# Autodesk Inventor assembly: CycloidalGearBoxAssemblyV1
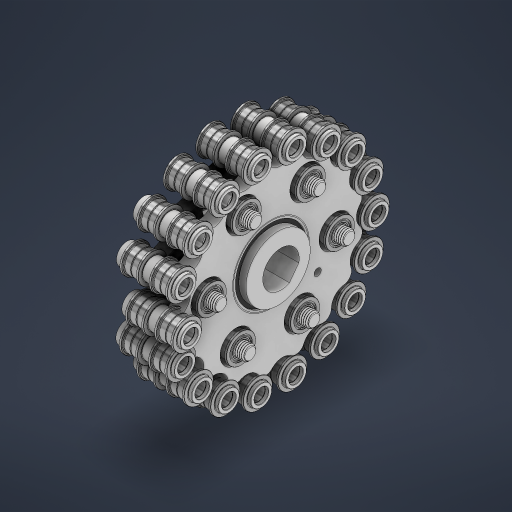
[picture p0: Inventor's stored thumbnail of the model, 512x512]
Saved by Autodesk Inventor 2024 (Build 280153000, 153)
## iProperties
Created: 2024-01-31
Part Number: CycloidalGearBoxAssemblyV1
Document SubType Name: Assembly
Designer: avsar
Author: avsar
## Documents named in this file (12)
- C:\Users\avsar\Documents\Inventor\RCR_Arm\Arm_V4\CycloidalGearBoxes\StageOneGearBox\CycloidalGearBoxAssemblyV1.iam
- C:\Users\avsar\Documents\Inventor\RCR_Arm\Arm_V4\CycloidalGearBoxes\StageOneGearBox\HousingFaceInput.ipt
- C:\Users\avsar\Documents\Inventor\RCR_Arm\Arm_V4\CycloidalGearBoxes\StageOneGearBox\Gearbox_MainBody.ipt
- C:\Users\avsar\Documents\Inventor\RCR_Arm\COTS\Motion\Bearings\Flanged Bearings\4x7x2.5mm Flanged Ball Bearing.ipt
- C:\Users\avsar\Documents\Inventor\RCR_Arm\COTS\ISO Standard Hardware\Spacers and Shims\4mm ID x 6mm OD Spacers\(1mm legnth) 4mm ID x 6mm OD Spacer.ipt
- C:\Users\avsar\Documents\Inventor\RCR_Arm\COTS\ISO Standard Hardware\Spacers and Shims\4mm ID x 6mm OD Spacers\(3mm legnth) 4mm ID x 6mm OD Spacer.ipt
- C:\Users\avsar\Documents\Inventor\RCR_Arm\Arm_V4\CycloidalGearBoxes\StageOneGearBox\RollerBearingShaft.ipt
- C:\Users\avsar\Documents\Inventor\RCR_Arm\Arm_V4\CycloidalGearBoxes\StageOneGearBox\CycloidalDisk.ipt
- C:\Users\avsar\Documents\Inventor\RCR_Arm\Arm_V4\CycloidalGearBoxes\StageOneGearBox\EccentricBearingShaft.ipt
- C:\Users\avsar\Documents\Inventor\RCR_Arm\COTS\Motion\Bearings\Standard Bearings\16mm ID x 22mm OD x 4mm Thickness Ball Bearing.ipt
- C:\Users\avsar\Documents\Inventor\RCR_Arm\COTS\ISO Standard Hardware\Screws\Sockethead Screws\Buttonhead Screws\M4 x 0.7mm\(M4 x 0.7 x 16) Sockethead Buttonhead Screw.ipt
- C:\Users\avsar\Documents\Inventor\RCR_Arm\Arm_V4\CycloidalGearBoxes\StageOneGearBox\HousingInputFaceSpacer.ipt
## Components (182 placed, 11 different names)
1. HousingFaceInput:1 — Mate:1, Mate:2, Mate:3, Mate:7, Mate:76, Mate:94, Mate:112, Mate:130, Mate:148, Mate:166, Mate:184, Mate:202, Mate:220, Mate:238, Mate:256, Mate:274, Mate:292, Mate:310, Mate:328, Mate:346, Mate:364
2. Gearbox_MainBody:1 — Mate:1, Mate:2, Mate:3
3. 4x7x2.5mm Flanged Ball Bearing:5 — Mate:10, Mate:11, Mate:12, Mate:13
4. RollerBearingShaft:2 — Mate:8, Mate:9, Mate:10, Mate:11
5. 4x7x2.5mm Flanged Ball Bearing:4 — Mate:7, Mate:8, Mate:9
6. (1mm legnth) 4mm ID x 6mm OD Spacer:2 — Mate:20, Mate:21
7. RollerBearingShaft:1 — Mate:16, Mate:17, Mate:18, Mate:19
8. 4x7x2.5mm Flanged Ball Bearing:2 — Mate:14, Mate:15, Mate:16, Mate:17
9. (3mm legnth) 4mm ID x 6mm OD Spacer:1 — Mate:12, Mate:13, Mate:14, Mate:15
10. 4x7x2.5mm Flanged Ball Bearing:1 — Mate:18, Mate:19, Mate:20, Mate:21
11. (1mm legnth) 4mm ID x 6mm OD Spacer:3 — Mate:76
12. 4x7x2.5mm Flanged Ball Bearing:6 — Mate:377
13. RollerBearingShaft:3
14. 4x7x2.5mm Flanged Ball Bearing:7
15. 4x7x2.5mm Flanged Ball Bearing:8
16. RollerBearingShaft:4
17. 4x7x2.5mm Flanged Ball Bearing:9
18. (3mm legnth) 4mm ID x 6mm OD Spacer:2
19. (1mm legnth) 4mm ID x 6mm OD Spacer:5 — Mate:94
20. 4x7x2.5mm Flanged Ball Bearing:10
21. RollerBearingShaft:5
22. 4x7x2.5mm Flanged Ball Bearing:11
23. 4x7x2.5mm Flanged Ball Bearing:12
24. RollerBearingShaft:6
25. 4x7x2.5mm Flanged Ball Bearing:13
26. (3mm legnth) 4mm ID x 6mm OD Spacer:3
27. (1mm legnth) 4mm ID x 6mm OD Spacer:7 — Mate:112
28. 4x7x2.5mm Flanged Ball Bearing:14
29. RollerBearingShaft:7
30. 4x7x2.5mm Flanged Ball Bearing:15 — Tangent:1
31. 4x7x2.5mm Flanged Ball Bearing:16
32. RollerBearingShaft:8
33. 4x7x2.5mm Flanged Ball Bearing:17
34. (3mm legnth) 4mm ID x 6mm OD Spacer:4
35. (1mm legnth) 4mm ID x 6mm OD Spacer:9
36. 4x7x2.5mm Flanged Ball Bearing:18
37. RollerBearingShaft:9
38. 4x7x2.5mm Flanged Ball Bearing:19
39. 4x7x2.5mm Flanged Ball Bearing:20 — Mate:130
40. RollerBearingShaft:10
41. 4x7x2.5mm Flanged Ball Bearing:21
42. (3mm legnth) 4mm ID x 6mm OD Spacer:5
43. (1mm legnth) 4mm ID x 6mm OD Spacer:11
44. 4x7x2.5mm Flanged Ball Bearing:22 — Mate:411, Mate:412
45. RollerBearingShaft:11
46. 4x7x2.5mm Flanged Ball Bearing:23
47. 4x7x2.5mm Flanged Ball Bearing:24 — Mate:148
48. RollerBearingShaft:12
49. 4x7x2.5mm Flanged Ball Bearing:25
50. (3mm legnth) 4mm ID x 6mm OD Spacer:6
51. (1mm legnth) 4mm ID x 6mm OD Spacer:13
52. 4x7x2.5mm Flanged Ball Bearing:26 — Mate:413, Mate:414
53. RollerBearingShaft:13
54. 4x7x2.5mm Flanged Ball Bearing:27 — Tangent:2
55. 4x7x2.5mm Flanged Ball Bearing:28 — Mate:166
56. RollerBearingShaft:14
57. 4x7x2.5mm Flanged Ball Bearing:29
58. (3mm legnth) 4mm ID x 6mm OD Spacer:7
59. (1mm legnth) 4mm ID x 6mm OD Spacer:15
60. 4x7x2.5mm Flanged Ball Bearing:30 — Mate:415, Mate:416
61. RollerBearingShaft:15
62. 4x7x2.5mm Flanged Ball Bearing:31
63. 4x7x2.5mm Flanged Ball Bearing:32 — Mate:184
64. RollerBearingShaft:16
65. 4x7x2.5mm Flanged Ball Bearing:33
66. (3mm legnth) 4mm ID x 6mm OD Spacer:8
67. (1mm legnth) 4mm ID x 6mm OD Spacer:17
68. 4x7x2.5mm Flanged Ball Bearing:34 — Mate:417, Mate:418
69. RollerBearingShaft:17
70. 4x7x2.5mm Flanged Ball Bearing:35
71. 4x7x2.5mm Flanged Ball Bearing:36 — Mate:202
72. RollerBearingShaft:18
73. 4x7x2.5mm Flanged Ball Bearing:37
74. (3mm legnth) 4mm ID x 6mm OD Spacer:9
75. (1mm legnth) 4mm ID x 6mm OD Spacer:19
76. 4x7x2.5mm Flanged Ball Bearing:38 — Mate:419, Mate:420
77. RollerBearingShaft:19
78. 4x7x2.5mm Flanged Ball Bearing:39
79. 4x7x2.5mm Flanged Ball Bearing:40 — Mate:220
80. RollerBearingShaft:20
81. 4x7x2.5mm Flanged Ball Bearing:41
82. (3mm legnth) 4mm ID x 6mm OD Spacer:10
83. (1mm legnth) 4mm ID x 6mm OD Spacer:21
84. 4x7x2.5mm Flanged Ball Bearing:42 — Mate:421, Mate:422
85. RollerBearingShaft:21
86. 4x7x2.5mm Flanged Ball Bearing:43
87. 4x7x2.5mm Flanged Ball Bearing:44 — Mate:238
88. RollerBearingShaft:22
89. 4x7x2.5mm Flanged Ball Bearing:45
90. (3mm legnth) 4mm ID x 6mm OD Spacer:11
91. (1mm legnth) 4mm ID x 6mm OD Spacer:23
92. 4x7x2.5mm Flanged Ball Bearing:46 — Mate:256, Mate:423, Mate:424
93. RollerBearingShaft:23
94. 4x7x2.5mm Flanged Ball Bearing:47
95. 4x7x2.5mm Flanged Ball Bearing:48
96. RollerBearingShaft:24
97. 4x7x2.5mm Flanged Ball Bearing:49
98. (3mm legnth) 4mm ID x 6mm OD Spacer:12
99. (1mm legnth) 4mm ID x 6mm OD Spacer:25
100. 4x7x2.5mm Flanged Ball Bearing:50 — Mate:425, Mate:426
101. RollerBearingShaft:25
102. 4x7x2.5mm Flanged Ball Bearing:51
103. 4x7x2.5mm Flanged Ball Bearing:52 — Mate:274
104. RollerBearingShaft:26
105. 4x7x2.5mm Flanged Ball Bearing:53
106. (3mm legnth) 4mm ID x 6mm OD Spacer:13
107. (1mm legnth) 4mm ID x 6mm OD Spacer:27
108. 4x7x2.5mm Flanged Ball Bearing:54 — Mate:427, Mate:428
109. RollerBearingShaft:27
110. 4x7x2.5mm Flanged Ball Bearing:55
111. 4x7x2.5mm Flanged Ball Bearing:56 — Mate:292
112. RollerBearingShaft:28
113. 4x7x2.5mm Flanged Ball Bearing:57
114. (3mm legnth) 4mm ID x 6mm OD Spacer:14
115. (1mm legnth) 4mm ID x 6mm OD Spacer:29
116. 4x7x2.5mm Flanged Ball Bearing:58 — Mate:429, Mate:430
117. RollerBearingShaft:29
118. 4x7x2.5mm Flanged Ball Bearing:59
119. 4x7x2.5mm Flanged Ball Bearing:60 — Mate:310
120. RollerBearingShaft:30
121. 4x7x2.5mm Flanged Ball Bearing:61
122. (3mm legnth) 4mm ID x 6mm OD Spacer:15
123. (1mm legnth) 4mm ID x 6mm OD Spacer:31
124. 4x7x2.5mm Flanged Ball Bearing:62 — Mate:431, Mate:432
125. RollerBearingShaft:31
126. 4x7x2.5mm Flanged Ball Bearing:63
127. 4x7x2.5mm Flanged Ball Bearing:64 — Mate:328
128. RollerBearingShaft:32
129. 4x7x2.5mm Flanged Ball Bearing:65
130. (3mm legnth) 4mm ID x 6mm OD Spacer:16
131. (1mm legnth) 4mm ID x 6mm OD Spacer:33
132. 4x7x2.5mm Flanged Ball Bearing:66 — Mate:433, Mate:434
133. RollerBearingShaft:33
134. 4x7x2.5mm Flanged Ball Bearing:67
135. 4x7x2.5mm Flanged Ball Bearing:68 — Mate:346
136. RollerBearingShaft:34
137. 4x7x2.5mm Flanged Ball Bearing:69
138. (3mm legnth) 4mm ID x 6mm OD Spacer:17
139. (1mm legnth) 4mm ID x 6mm OD Spacer:35
140. 4x7x2.5mm Flanged Ball Bearing:70 — Mate:435, Mate:436
141. RollerBearingShaft:35
142. 4x7x2.5mm Flanged Ball Bearing:71
143. 4x7x2.5mm Flanged Ball Bearing:72 — Mate:364, Tangent:15
144. RollerBearingShaft:36
145. 4x7x2.5mm Flanged Ball Bearing:73
146. (3mm legnth) 4mm ID x 6mm OD Spacer:18
147. 16mm ID x 22mm OD x 4mm Thickness Ball Bearing:3 — Flush:5, Mate:375, Mate:378
148. EccentricBearingShaft:2 — Mate:372, Mate:373, Mate:378
149. CycloidalDisk:3 — Mate:374, Flush:4, Mate:377, Tangent:1, Tangent:2, Mate:382, Tangent:4, Mate:387, Tangent:6, Mate:395, Mate:396, Mate:397, Mate:398, Tangent:11, Tangent:12, Tangent:13, Tangent:14
150. CycloidalDisk:4 — Flush:5, Mate:375, Mate:379, Tangent:3, Mate:386, Tangent:5, Mate:391, Tangent:7, Mate:392, Mate:393, Mate:394, Tangent:8, Tangent:9, Tangent:10, Tangent:15
151. 16mm ID x 22mm OD x 4mm Thickness Ball Bearing:4 — Mate:372, Mate:373, Mate:374, Flush:4
152. 4x7x2.5mm Flanged Ball Bearing:74 — Mate:379, Tangent:3, Mate:385
153. 4x7x2.5mm Flanged Ball Bearing:75 — Mate:382, Tangent:4, Mate:383, Mate:384
154. (M4 x 0.7 x 16) Sockethead Buttonhead Screw:1 — Mate:383, Mate:384, Mate:385
155. 4x7x2.5mm Flanged Ball Bearing:76 — Mate:386, Tangent:5, Mate:390
156. 4x7x2.5mm Flanged Ball Bearing:77 — Mate:387, Tangent:6, Mate:388, Mate:389
157. (M4 x 0.7 x 16) Sockethead Buttonhead Screw:2 — Mate:388, Mate:389, Mate:390
158. 4x7x2.5mm Flanged Ball Bearing:78 — Mate:391, Tangent:7, Mate:408
159. 4x7x2.5mm Flanged Ball Bearing:79 — Mate:392, Tangent:8, Mate:409
160. 4x7x2.5mm Flanged Ball Bearing:80 — Mate:393, Tangent:9, Mate:410
161. 4x7x2.5mm Flanged Ball Bearing:81 — Mate:394, Tangent:10, Mate:407
162. 4x7x2.5mm Flanged Ball Bearing:82 — Mate:395, Tangent:11, Mate:405, Mate:406
163. 4x7x2.5mm Flanged Ball Bearing:83 — Mate:396, Tangent:12, Mate:403, Mate:404
164. 4x7x2.5mm Flanged Ball Bearing:84 — Mate:397, Tangent:13, Mate:401, Mate:402
165. 4x7x2.5mm Flanged Ball Bearing:85 — Mate:398, Tangent:14, Mate:399, Mate:400
166. (M4 x 0.7 x 16) Sockethead Buttonhead Screw:3 — Mate:399, Mate:400, Mate:408
167. (M4 x 0.7 x 16) Sockethead Buttonhead Screw:4 — Mate:401, Mate:402, Mate:409
168. (M4 x 0.7 x 16) Sockethead Buttonhead Screw:5 — Mate:403, Mate:404, Mate:410
169. (M4 x 0.7 x 16) Sockethead Buttonhead Screw:6 — Mate:405, Mate:406, Mate:407
170. HousingInputFaceSpacer:1 — Mate:411, Mate:412
171. HousingInputFaceSpacer:2 — Mate:413, Mate:414
172. HousingInputFaceSpacer:3 — Mate:415, Mate:416
173. HousingInputFaceSpacer:4 — Mate:417, Mate:418
174. HousingInputFaceSpacer:5 — Mate:419, Mate:420
175. HousingInputFaceSpacer:6 — Mate:421, Mate:422
176. HousingInputFaceSpacer:7 — Mate:423, Mate:424
177. HousingInputFaceSpacer:8 — Mate:425, Mate:426
178. HousingInputFaceSpacer:9 — Mate:427, Mate:428
179. HousingInputFaceSpacer:10 — Mate:429, Mate:430
180. HousingInputFaceSpacer:11 — Mate:431, Mate:432
181. HousingInputFaceSpacer:12 — Mate:433, Mate:434
182. HousingInputFaceSpacer:13 — Mate:435, Mate:436
## Relationships (353: Mate 336, Tangent 15, Flush 2)
- Mate:1: HousingFaceInput:1 ↔ Gearbox_MainBody:1
- Mate:2: HousingFaceInput:1 ↔ Gearbox_MainBody:1
- Mate:3: HousingFaceInput:1 ↔ Gearbox_MainBody:1
- Mate:7: HousingFaceInput:1 ↔ 4x7x2.5mm Flanged Ball Bearing:4
- Mate:8: RollerBearingShaft:2 ↔ 4x7x2.5mm Flanged Ball Bearing:4
- Mate:9: RollerBearingShaft:2 ↔ 4x7x2.5mm Flanged Ball Bearing:4
- Mate:10: 4x7x2.5mm Flanged Ball Bearing:5 ↔ RollerBearingShaft:2
- Mate:11: 4x7x2.5mm Flanged Ball Bearing:5 ↔ RollerBearingShaft:2
- Mate:12: 4x7x2.5mm Flanged Ball Bearing:5 ↔ (3mm legnth) 4mm ID x 6mm OD Spacer:1
- Mate:13: 4x7x2.5mm Flanged Ball Bearing:5 ↔ (3mm legnth) 4mm ID x 6mm OD Spacer:1
- Mate:14: 4x7x2.5mm Flanged Ball Bearing:2 ↔ (3mm legnth) 4mm ID x 6mm OD Spacer:1
- Mate:15: 4x7x2.5mm Flanged Ball Bearing:2 ↔ (3mm legnth) 4mm ID x 6mm OD Spacer:1
- Mate:16: RollerBearingShaft:1 ↔ 4x7x2.5mm Flanged Ball Bearing:2
- Mate:17: RollerBearingShaft:1 ↔ 4x7x2.5mm Flanged Ball Bearing:2
- Mate:18: RollerBearingShaft:1 ↔ 4x7x2.5mm Flanged Ball Bearing:1
- Mate:19: RollerBearingShaft:1 ↔ 4x7x2.5mm Flanged Ball Bearing:1
- Mate:20: (1mm legnth) 4mm ID x 6mm OD Spacer:2 ↔ 4x7x2.5mm Flanged Ball Bearing:1
- Mate:21: (1mm legnth) 4mm ID x 6mm OD Spacer:2 ↔ 4x7x2.5mm Flanged Ball Bearing:1
- [Mate]: (1mm legnth) 4mm ID x 6mm OD Spacer:3 ↔ 4x7x2.5mm Flanged Ball Bearing:8
- [Mate]: 4x7x2.5mm Flanged Ball Bearing:8 ↔ RollerBearingShaft:4
- [Mate]: 4x7x2.5mm Flanged Ball Bearing:8 ↔ RollerBearingShaft:4
- [Mate]: RollerBearingShaft:4 ↔ 4x7x2.5mm Flanged Ball Bearing:9
- [Mate]: RollerBearingShaft:4 ↔ 4x7x2.5mm Flanged Ball Bearing:9
- [Mate]: 4x7x2.5mm Flanged Ball Bearing:9 ↔ (3mm legnth) 4mm ID x 6mm OD Spacer:2
- [Mate]: 4x7x2.5mm Flanged Ball Bearing:9 ↔ (3mm legnth) 4mm ID x 6mm OD Spacer:2
- [Mate]: 4x7x2.5mm Flanged Ball Bearing:7 ↔ (3mm legnth) 4mm ID x 6mm OD Spacer:2
- [Mate]: 4x7x2.5mm Flanged Ball Bearing:7 ↔ (3mm legnth) 4mm ID x 6mm OD Spacer:2
- [Mate]: RollerBearingShaft:3 ↔ 4x7x2.5mm Flanged Ball Bearing:7
- [Mate]: RollerBearingShaft:3 ↔ 4x7x2.5mm Flanged Ball Bearing:7
- [Mate]: 4x7x2.5mm Flanged Ball Bearing:6 ↔ RollerBearingShaft:3
- [Mate]: 4x7x2.5mm Flanged Ball Bearing:6 ↔ RollerBearingShaft:3
- [Mate]: (1mm legnth) 4mm ID x 6mm OD Spacer:3 ↔ 4x7x2.5mm Flanged Ball Bearing:8
- Mate:76: HousingFaceInput:1 ↔ (1mm legnth) 4mm ID x 6mm OD Spacer:3
- [Mate]: (1mm legnth) 4mm ID x 6mm OD Spacer:5 ↔ 4x7x2.5mm Flanged Ball Bearing:12
- [Mate]: 4x7x2.5mm Flanged Ball Bearing:12 ↔ RollerBearingShaft:6
- [Mate]: 4x7x2.5mm Flanged Ball Bearing:12 ↔ RollerBearingShaft:6
- [Mate]: RollerBearingShaft:6 ↔ 4x7x2.5mm Flanged Ball Bearing:13
- [Mate]: RollerBearingShaft:6 ↔ 4x7x2.5mm Flanged Ball Bearing:13
- [Mate]: 4x7x2.5mm Flanged Ball Bearing:13 ↔ (3mm legnth) 4mm ID x 6mm OD Spacer:3
- [Mate]: 4x7x2.5mm Flanged Ball Bearing:13 ↔ (3mm legnth) 4mm ID x 6mm OD Spacer:3
- [Mate]: 4x7x2.5mm Flanged Ball Bearing:11 ↔ (3mm legnth) 4mm ID x 6mm OD Spacer:3
- [Mate]: 4x7x2.5mm Flanged Ball Bearing:11 ↔ (3mm legnth) 4mm ID x 6mm OD Spacer:3
- [Mate]: RollerBearingShaft:5 ↔ 4x7x2.5mm Flanged Ball Bearing:11
- [Mate]: RollerBearingShaft:5 ↔ 4x7x2.5mm Flanged Ball Bearing:11
- [Mate]: 4x7x2.5mm Flanged Ball Bearing:10 ↔ RollerBearingShaft:5
- [Mate]: 4x7x2.5mm Flanged Ball Bearing:10 ↔ RollerBearingShaft:5
- [Mate]: (1mm legnth) 4mm ID x 6mm OD Spacer:5 ↔ 4x7x2.5mm Flanged Ball Bearing:12
- Mate:94: HousingFaceInput:1 ↔ (1mm legnth) 4mm ID x 6mm OD Spacer:5
- [Mate]: (1mm legnth) 4mm ID x 6mm OD Spacer:7 ↔ 4x7x2.5mm Flanged Ball Bearing:16
- [Mate]: 4x7x2.5mm Flanged Ball Bearing:16 ↔ RollerBearingShaft:8
- [Mate]: 4x7x2.5mm Flanged Ball Bearing:16 ↔ RollerBearingShaft:8
- [Mate]: RollerBearingShaft:8 ↔ 4x7x2.5mm Flanged Ball Bearing:17
- [Mate]: RollerBearingShaft:8 ↔ 4x7x2.5mm Flanged Ball Bearing:17
- [Mate]: 4x7x2.5mm Flanged Ball Bearing:17 ↔ (3mm legnth) 4mm ID x 6mm OD Spacer:4
- [Mate]: 4x7x2.5mm Flanged Ball Bearing:17 ↔ (3mm legnth) 4mm ID x 6mm OD Spacer:4
- [Mate]: 4x7x2.5mm Flanged Ball Bearing:15 ↔ (3mm legnth) 4mm ID x 6mm OD Spacer:4
- [Mate]: 4x7x2.5mm Flanged Ball Bearing:15 ↔ (3mm legnth) 4mm ID x 6mm OD Spacer:4
- [Mate]: RollerBearingShaft:7 ↔ 4x7x2.5mm Flanged Ball Bearing:15
- [Mate]: RollerBearingShaft:7 ↔ 4x7x2.5mm Flanged Ball Bearing:15
- [Mate]: 4x7x2.5mm Flanged Ball Bearing:14 ↔ RollerBearingShaft:7
- [Mate]: 4x7x2.5mm Flanged Ball Bearing:14 ↔ RollerBearingShaft:7
- [Mate]: (1mm legnth) 4mm ID x 6mm OD Spacer:7 ↔ 4x7x2.5mm Flanged Ball Bearing:16
- Mate:112: HousingFaceInput:1 ↔ (1mm legnth) 4mm ID x 6mm OD Spacer:7
- [Mate]: (1mm legnth) 4mm ID x 6mm OD Spacer:9 ↔ 4x7x2.5mm Flanged Ball Bearing:20
- [Mate]: 4x7x2.5mm Flanged Ball Bearing:20 ↔ RollerBearingShaft:10
- [Mate]: 4x7x2.5mm Flanged Ball Bearing:20 ↔ RollerBearingShaft:10
- [Mate]: RollerBearingShaft:10 ↔ 4x7x2.5mm Flanged Ball Bearing:21
- [Mate]: RollerBearingShaft:10 ↔ 4x7x2.5mm Flanged Ball Bearing:21
- [Mate]: 4x7x2.5mm Flanged Ball Bearing:21 ↔ (3mm legnth) 4mm ID x 6mm OD Spacer:5
- [Mate]: 4x7x2.5mm Flanged Ball Bearing:21 ↔ (3mm legnth) 4mm ID x 6mm OD Spacer:5
- [Mate]: 4x7x2.5mm Flanged Ball Bearing:19 ↔ (3mm legnth) 4mm ID x 6mm OD Spacer:5
- [Mate]: 4x7x2.5mm Flanged Ball Bearing:19 ↔ (3mm legnth) 4mm ID x 6mm OD Spacer:5
- [Mate]: RollerBearingShaft:9 ↔ 4x7x2.5mm Flanged Ball Bearing:19
- [Mate]: RollerBearingShaft:9 ↔ 4x7x2.5mm Flanged Ball Bearing:19
- [Mate]: 4x7x2.5mm Flanged Ball Bearing:18 ↔ RollerBearingShaft:9
- [Mate]: 4x7x2.5mm Flanged Ball Bearing:18 ↔ RollerBearingShaft:9
- [Mate]: (1mm legnth) 4mm ID x 6mm OD Spacer:9 ↔ 4x7x2.5mm Flanged Ball Bearing:20
- Mate:130: HousingFaceInput:1 ↔ 4x7x2.5mm Flanged Ball Bearing:20
- [Mate]: (1mm legnth) 4mm ID x 6mm OD Spacer:11 ↔ 4x7x2.5mm Flanged Ball Bearing:24
- [Mate]: 4x7x2.5mm Flanged Ball Bearing:24 ↔ RollerBearingShaft:12
- [Mate]: 4x7x2.5mm Flanged Ball Bearing:24 ↔ RollerBearingShaft:12
- [Mate]: RollerBearingShaft:12 ↔ 4x7x2.5mm Flanged Ball Bearing:25
- [Mate]: RollerBearingShaft:12 ↔ 4x7x2.5mm Flanged Ball Bearing:25
- [Mate]: 4x7x2.5mm Flanged Ball Bearing:25 ↔ (3mm legnth) 4mm ID x 6mm OD Spacer:6
- [Mate]: 4x7x2.5mm Flanged Ball Bearing:25 ↔ (3mm legnth) 4mm ID x 6mm OD Spacer:6
- [Mate]: 4x7x2.5mm Flanged Ball Bearing:23 ↔ (3mm legnth) 4mm ID x 6mm OD Spacer:6
- [Mate]: 4x7x2.5mm Flanged Ball Bearing:23 ↔ (3mm legnth) 4mm ID x 6mm OD Spacer:6
- [Mate]: RollerBearingShaft:11 ↔ 4x7x2.5mm Flanged Ball Bearing:23
- [Mate]: RollerBearingShaft:11 ↔ 4x7x2.5mm Flanged Ball Bearing:23
- [Mate]: 4x7x2.5mm Flanged Ball Bearing:22 ↔ RollerBearingShaft:11
- [Mate]: 4x7x2.5mm Flanged Ball Bearing:22 ↔ RollerBearingShaft:11
- [Mate]: (1mm legnth) 4mm ID x 6mm OD Spacer:11 ↔ 4x7x2.5mm Flanged Ball Bearing:24
- Mate:148: HousingFaceInput:1 ↔ 4x7x2.5mm Flanged Ball Bearing:24
- [Mate]: (1mm legnth) 4mm ID x 6mm OD Spacer:13 ↔ 4x7x2.5mm Flanged Ball Bearing:28
- [Mate]: 4x7x2.5mm Flanged Ball Bearing:28 ↔ RollerBearingShaft:14
- [Mate]: 4x7x2.5mm Flanged Ball Bearing:28 ↔ RollerBearingShaft:14
- [Mate]: RollerBearingShaft:14 ↔ 4x7x2.5mm Flanged Ball Bearing:29
- [Mate]: RollerBearingShaft:14 ↔ 4x7x2.5mm Flanged Ball Bearing:29
- [Mate]: 4x7x2.5mm Flanged Ball Bearing:29 ↔ (3mm legnth) 4mm ID x 6mm OD Spacer:7
- [Mate]: 4x7x2.5mm Flanged Ball Bearing:29 ↔ (3mm legnth) 4mm ID x 6mm OD Spacer:7
- [Mate]: 4x7x2.5mm Flanged Ball Bearing:27 ↔ (3mm legnth) 4mm ID x 6mm OD Spacer:7
- [Mate]: 4x7x2.5mm Flanged Ball Bearing:27 ↔ (3mm legnth) 4mm ID x 6mm OD Spacer:7
- [Mate]: RollerBearingShaft:13 ↔ 4x7x2.5mm Flanged Ball Bearing:27
- [Mate]: RollerBearingShaft:13 ↔ 4x7x2.5mm Flanged Ball Bearing:27
- [Mate]: 4x7x2.5mm Flanged Ball Bearing:26 ↔ RollerBearingShaft:13
- [Mate]: 4x7x2.5mm Flanged Ball Bearing:26 ↔ RollerBearingShaft:13
- [Mate]: (1mm legnth) 4mm ID x 6mm OD Spacer:13 ↔ 4x7x2.5mm Flanged Ball Bearing:28
- Mate:166: HousingFaceInput:1 ↔ 4x7x2.5mm Flanged Ball Bearing:28
- [Mate]: (1mm legnth) 4mm ID x 6mm OD Spacer:15 ↔ 4x7x2.5mm Flanged Ball Bearing:32
- [Mate]: 4x7x2.5mm Flanged Ball Bearing:32 ↔ RollerBearingShaft:16
- [Mate]: 4x7x2.5mm Flanged Ball Bearing:32 ↔ RollerBearingShaft:16
- [Mate]: RollerBearingShaft:16 ↔ 4x7x2.5mm Flanged Ball Bearing:33
- [Mate]: RollerBearingShaft:16 ↔ 4x7x2.5mm Flanged Ball Bearing:33
- [Mate]: 4x7x2.5mm Flanged Ball Bearing:33 ↔ (3mm legnth) 4mm ID x 6mm OD Spacer:8
- [Mate]: 4x7x2.5mm Flanged Ball Bearing:33 ↔ (3mm legnth) 4mm ID x 6mm OD Spacer:8
- [Mate]: 4x7x2.5mm Flanged Ball Bearing:31 ↔ (3mm legnth) 4mm ID x 6mm OD Spacer:8
- [Mate]: 4x7x2.5mm Flanged Ball Bearing:31 ↔ (3mm legnth) 4mm ID x 6mm OD Spacer:8
- [Mate]: RollerBearingShaft:15 ↔ 4x7x2.5mm Flanged Ball Bearing:31
- [Mate]: RollerBearingShaft:15 ↔ 4x7x2.5mm Flanged Ball Bearing:31
- [Mate]: 4x7x2.5mm Flanged Ball Bearing:30 ↔ RollerBearingShaft:15
- [Mate]: 4x7x2.5mm Flanged Ball Bearing:30 ↔ RollerBearingShaft:15
- [Mate]: (1mm legnth) 4mm ID x 6mm OD Spacer:15 ↔ 4x7x2.5mm Flanged Ball Bearing:32
- Mate:184: HousingFaceInput:1 ↔ 4x7x2.5mm Flanged Ball Bearing:32
- [Mate]: (1mm legnth) 4mm ID x 6mm OD Spacer:17 ↔ 4x7x2.5mm Flanged Ball Bearing:36
- [Mate]: 4x7x2.5mm Flanged Ball Bearing:36 ↔ RollerBearingShaft:18
- [Mate]: 4x7x2.5mm Flanged Ball Bearing:36 ↔ RollerBearingShaft:18
- [Mate]: RollerBearingShaft:18 ↔ 4x7x2.5mm Flanged Ball Bearing:37
- [Mate]: RollerBearingShaft:18 ↔ 4x7x2.5mm Flanged Ball Bearing:37
- [Mate]: 4x7x2.5mm Flanged Ball Bearing:37 ↔ (3mm legnth) 4mm ID x 6mm OD Spacer:9
- [Mate]: 4x7x2.5mm Flanged Ball Bearing:37 ↔ (3mm legnth) 4mm ID x 6mm OD Spacer:9
- [Mate]: 4x7x2.5mm Flanged Ball Bearing:35 ↔ (3mm legnth) 4mm ID x 6mm OD Spacer:9
- [Mate]: 4x7x2.5mm Flanged Ball Bearing:35 ↔ (3mm legnth) 4mm ID x 6mm OD Spacer:9
- [Mate]: RollerBearingShaft:17 ↔ 4x7x2.5mm Flanged Ball Bearing:35
- [Mate]: RollerBearingShaft:17 ↔ 4x7x2.5mm Flanged Ball Bearing:35
- [Mate]: 4x7x2.5mm Flanged Ball Bearing:34 ↔ RollerBearingShaft:17
- [Mate]: 4x7x2.5mm Flanged Ball Bearing:34 ↔ RollerBearingShaft:17
- [Mate]: (1mm legnth) 4mm ID x 6mm OD Spacer:17 ↔ 4x7x2.5mm Flanged Ball Bearing:36
- Mate:202: HousingFaceInput:1 ↔ 4x7x2.5mm Flanged Ball Bearing:36
- [Mate]: (1mm legnth) 4mm ID x 6mm OD Spacer:19 ↔ 4x7x2.5mm Flanged Ball Bearing:40
- [Mate]: 4x7x2.5mm Flanged Ball Bearing:40 ↔ RollerBearingShaft:20
- [Mate]: 4x7x2.5mm Flanged Ball Bearing:40 ↔ RollerBearingShaft:20
- [Mate]: RollerBearingShaft:20 ↔ 4x7x2.5mm Flanged Ball Bearing:41
- [Mate]: RollerBearingShaft:20 ↔ 4x7x2.5mm Flanged Ball Bearing:41
- [Mate]: 4x7x2.5mm Flanged Ball Bearing:41 ↔ (3mm legnth) 4mm ID x 6mm OD Spacer:10
- [Mate]: 4x7x2.5mm Flanged Ball Bearing:41 ↔ (3mm legnth) 4mm ID x 6mm OD Spacer:10
- [Mate]: 4x7x2.5mm Flanged Ball Bearing:39 ↔ (3mm legnth) 4mm ID x 6mm OD Spacer:10
- [Mate]: 4x7x2.5mm Flanged Ball Bearing:39 ↔ (3mm legnth) 4mm ID x 6mm OD Spacer:10
- [Mate]: RollerBearingShaft:19 ↔ 4x7x2.5mm Flanged Ball Bearing:39
- [Mate]: RollerBearingShaft:19 ↔ 4x7x2.5mm Flanged Ball Bearing:39
- [Mate]: 4x7x2.5mm Flanged Ball Bearing:38 ↔ RollerBearingShaft:19
- [Mate]: 4x7x2.5mm Flanged Ball Bearing:38 ↔ RollerBearingShaft:19
- [Mate]: (1mm legnth) 4mm ID x 6mm OD Spacer:19 ↔ 4x7x2.5mm Flanged Ball Bearing:40
- Mate:220: HousingFaceInput:1 ↔ 4x7x2.5mm Flanged Ball Bearing:40
- [Mate]: (1mm legnth) 4mm ID x 6mm OD Spacer:21 ↔ 4x7x2.5mm Flanged Ball Bearing:44
- [Mate]: 4x7x2.5mm Flanged Ball Bearing:44 ↔ RollerBearingShaft:22
- [Mate]: 4x7x2.5mm Flanged Ball Bearing:44 ↔ RollerBearingShaft:22
- [Mate]: RollerBearingShaft:22 ↔ 4x7x2.5mm Flanged Ball Bearing:45
- [Mate]: RollerBearingShaft:22 ↔ 4x7x2.5mm Flanged Ball Bearing:45
- [Mate]: 4x7x2.5mm Flanged Ball Bearing:45 ↔ (3mm legnth) 4mm ID x 6mm OD Spacer:11
- [Mate]: 4x7x2.5mm Flanged Ball Bearing:45 ↔ (3mm legnth) 4mm ID x 6mm OD Spacer:11
- [Mate]: 4x7x2.5mm Flanged Ball Bearing:43 ↔ (3mm legnth) 4mm ID x 6mm OD Spacer:11
- [Mate]: 4x7x2.5mm Flanged Ball Bearing:43 ↔ (3mm legnth) 4mm ID x 6mm OD Spacer:11
- [Mate]: RollerBearingShaft:21 ↔ 4x7x2.5mm Flanged Ball Bearing:43
- [Mate]: RollerBearingShaft:21 ↔ 4x7x2.5mm Flanged Ball Bearing:43
- [Mate]: 4x7x2.5mm Flanged Ball Bearing:42 ↔ RollerBearingShaft:21
- [Mate]: 4x7x2.5mm Flanged Ball Bearing:42 ↔ RollerBearingShaft:21
- [Mate]: (1mm legnth) 4mm ID x 6mm OD Spacer:21 ↔ 4x7x2.5mm Flanged Ball Bearing:44
- Mate:238: HousingFaceInput:1 ↔ 4x7x2.5mm Flanged Ball Bearing:44
- [Mate]: (1mm legnth) 4mm ID x 6mm OD Spacer:23 ↔ 4x7x2.5mm Flanged Ball Bearing:48
- [Mate]: 4x7x2.5mm Flanged Ball Bearing:48 ↔ RollerBearingShaft:24
- [Mate]: 4x7x2.5mm Flanged Ball Bearing:48 ↔ RollerBearingShaft:24
- [Mate]: RollerBearingShaft:24 ↔ 4x7x2.5mm Flanged Ball Bearing:49
- [Mate]: RollerBearingShaft:24 ↔ 4x7x2.5mm Flanged Ball Bearing:49
- [Mate]: 4x7x2.5mm Flanged Ball Bearing:49 ↔ (3mm legnth) 4mm ID x 6mm OD Spacer:12
- [Mate]: 4x7x2.5mm Flanged Ball Bearing:49 ↔ (3mm legnth) 4mm ID x 6mm OD Spacer:12
- [Mate]: 4x7x2.5mm Flanged Ball Bearing:47 ↔ (3mm legnth) 4mm ID x 6mm OD Spacer:12
- [Mate]: 4x7x2.5mm Flanged Ball Bearing:47 ↔ (3mm legnth) 4mm ID x 6mm OD Spacer:12
- [Mate]: RollerBearingShaft:23 ↔ 4x7x2.5mm Flanged Ball Bearing:47
- [Mate]: RollerBearingShaft:23 ↔ 4x7x2.5mm Flanged Ball Bearing:47
- [Mate]: 4x7x2.5mm Flanged Ball Bearing:46 ↔ RollerBearingShaft:23
- [Mate]: 4x7x2.5mm Flanged Ball Bearing:46 ↔ RollerBearingShaft:23
- [Mate]: (1mm legnth) 4mm ID x 6mm OD Spacer:23 ↔ 4x7x2.5mm Flanged Ball Bearing:48
- Mate:256: HousingFaceInput:1 ↔ 4x7x2.5mm Flanged Ball Bearing:46
- [Mate]: (1mm legnth) 4mm ID x 6mm OD Spacer:25 ↔ 4x7x2.5mm Flanged Ball Bearing:52
- [Mate]: 4x7x2.5mm Flanged Ball Bearing:52 ↔ RollerBearingShaft:26
- [Mate]: 4x7x2.5mm Flanged Ball Bearing:52 ↔ RollerBearingShaft:26
- [Mate]: RollerBearingShaft:26 ↔ 4x7x2.5mm Flanged Ball Bearing:53
- [Mate]: RollerBearingShaft:26 ↔ 4x7x2.5mm Flanged Ball Bearing:53
- [Mate]: 4x7x2.5mm Flanged Ball Bearing:53 ↔ (3mm legnth) 4mm ID x 6mm OD Spacer:13
- [Mate]: 4x7x2.5mm Flanged Ball Bearing:53 ↔ (3mm legnth) 4mm ID x 6mm OD Spacer:13
- [Mate]: 4x7x2.5mm Flanged Ball Bearing:51 ↔ (3mm legnth) 4mm ID x 6mm OD Spacer:13
- [Mate]: 4x7x2.5mm Flanged Ball Bearing:51 ↔ (3mm legnth) 4mm ID x 6mm OD Spacer:13
- [Mate]: RollerBearingShaft:25 ↔ 4x7x2.5mm Flanged Ball Bearing:51
- [Mate]: RollerBearingShaft:25 ↔ 4x7x2.5mm Flanged Ball Bearing:51
- [Mate]: 4x7x2.5mm Flanged Ball Bearing:50 ↔ RollerBearingShaft:25
- [Mate]: 4x7x2.5mm Flanged Ball Bearing:50 ↔ RollerBearingShaft:25
- [Mate]: (1mm legnth) 4mm ID x 6mm OD Spacer:25 ↔ 4x7x2.5mm Flanged Ball Bearing:52
- Mate:274: HousingFaceInput:1 ↔ 4x7x2.5mm Flanged Ball Bearing:52
- [Mate]: (1mm legnth) 4mm ID x 6mm OD Spacer:27 ↔ 4x7x2.5mm Flanged Ball Bearing:56
- [Mate]: 4x7x2.5mm Flanged Ball Bearing:56 ↔ RollerBearingShaft:28
- [Mate]: 4x7x2.5mm Flanged Ball Bearing:56 ↔ RollerBearingShaft:28
- [Mate]: RollerBearingShaft:28 ↔ 4x7x2.5mm Flanged Ball Bearing:57
- [Mate]: RollerBearingShaft:28 ↔ 4x7x2.5mm Flanged Ball Bearing:57
- [Mate]: 4x7x2.5mm Flanged Ball Bearing:57 ↔ (3mm legnth) 4mm ID x 6mm OD Spacer:14
- [Mate]: 4x7x2.5mm Flanged Ball Bearing:57 ↔ (3mm legnth) 4mm ID x 6mm OD Spacer:14
- [Mate]: 4x7x2.5mm Flanged Ball Bearing:55 ↔ (3mm legnth) 4mm ID x 6mm OD Spacer:14
- [Mate]: 4x7x2.5mm Flanged Ball Bearing:55 ↔ (3mm legnth) 4mm ID x 6mm OD Spacer:14
- [Mate]: RollerBearingShaft:27 ↔ 4x7x2.5mm Flanged Ball Bearing:55
- [Mate]: RollerBearingShaft:27 ↔ 4x7x2.5mm Flanged Ball Bearing:55
- [Mate]: 4x7x2.5mm Flanged Ball Bearing:54 ↔ RollerBearingShaft:27
- [Mate]: 4x7x2.5mm Flanged Ball Bearing:54 ↔ RollerBearingShaft:27
- [Mate]: (1mm legnth) 4mm ID x 6mm OD Spacer:27 ↔ 4x7x2.5mm Flanged Ball Bearing:56
- Mate:292: HousingFaceInput:1 ↔ 4x7x2.5mm Flanged Ball Bearing:56
- [Mate]: (1mm legnth) 4mm ID x 6mm OD Spacer:29 ↔ 4x7x2.5mm Flanged Ball Bearing:60
- [Mate]: 4x7x2.5mm Flanged Ball Bearing:60 ↔ RollerBearingShaft:30
- [Mate]: 4x7x2.5mm Flanged Ball Bearing:60 ↔ RollerBearingShaft:30
- [Mate]: RollerBearingShaft:30 ↔ 4x7x2.5mm Flanged Ball Bearing:61
- [Mate]: RollerBearingShaft:30 ↔ 4x7x2.5mm Flanged Ball Bearing:61
- [Mate]: 4x7x2.5mm Flanged Ball Bearing:61 ↔ (3mm legnth) 4mm ID x 6mm OD Spacer:15
- [Mate]: 4x7x2.5mm Flanged Ball Bearing:61 ↔ (3mm legnth) 4mm ID x 6mm OD Spacer:15
- [Mate]: 4x7x2.5mm Flanged Ball Bearing:59 ↔ (3mm legnth) 4mm ID x 6mm OD Spacer:15
- [Mate]: 4x7x2.5mm Flanged Ball Bearing:59 ↔ (3mm legnth) 4mm ID x 6mm OD Spacer:15
- [Mate]: RollerBearingShaft:29 ↔ 4x7x2.5mm Flanged Ball Bearing:59
- [Mate]: RollerBearingShaft:29 ↔ 4x7x2.5mm Flanged Ball Bearing:59
- [Mate]: 4x7x2.5mm Flanged Ball Bearing:58 ↔ RollerBearingShaft:29
- [Mate]: 4x7x2.5mm Flanged Ball Bearing:58 ↔ RollerBearingShaft:29
- [Mate]: (1mm legnth) 4mm ID x 6mm OD Spacer:29 ↔ 4x7x2.5mm Flanged Ball Bearing:60
- Mate:310: HousingFaceInput:1 ↔ 4x7x2.5mm Flanged Ball Bearing:60
- [Mate]: (1mm legnth) 4mm ID x 6mm OD Spacer:31 ↔ 4x7x2.5mm Flanged Ball Bearing:64
- [Mate]: 4x7x2.5mm Flanged Ball Bearing:64 ↔ RollerBearingShaft:32
- [Mate]: 4x7x2.5mm Flanged Ball Bearing:64 ↔ RollerBearingShaft:32
- [Mate]: RollerBearingShaft:32 ↔ 4x7x2.5mm Flanged Ball Bearing:65
- [Mate]: RollerBearingShaft:32 ↔ 4x7x2.5mm Flanged Ball Bearing:65
- [Mate]: 4x7x2.5mm Flanged Ball Bearing:65 ↔ (3mm legnth) 4mm ID x 6mm OD Spacer:16
- [Mate]: 4x7x2.5mm Flanged Ball Bearing:65 ↔ (3mm legnth) 4mm ID x 6mm OD Spacer:16
- [Mate]: 4x7x2.5mm Flanged Ball Bearing:63 ↔ (3mm legnth) 4mm ID x 6mm OD Spacer:16
- [Mate]: 4x7x2.5mm Flanged Ball Bearing:63 ↔ (3mm legnth) 4mm ID x 6mm OD Spacer:16
- [Mate]: RollerBearingShaft:31 ↔ 4x7x2.5mm Flanged Ball Bearing:63
- [Mate]: RollerBearingShaft:31 ↔ 4x7x2.5mm Flanged Ball Bearing:63
- [Mate]: 4x7x2.5mm Flanged Ball Bearing:62 ↔ RollerBearingShaft:31
- [Mate]: 4x7x2.5mm Flanged Ball Bearing:62 ↔ RollerBearingShaft:31
- [Mate]: (1mm legnth) 4mm ID x 6mm OD Spacer:31 ↔ 4x7x2.5mm Flanged Ball Bearing:64
- Mate:328: HousingFaceInput:1 ↔ 4x7x2.5mm Flanged Ball Bearing:64
- [Mate]: (1mm legnth) 4mm ID x 6mm OD Spacer:33 ↔ 4x7x2.5mm Flanged Ball Bearing:68
- [Mate]: 4x7x2.5mm Flanged Ball Bearing:68 ↔ RollerBearingShaft:34
- [Mate]: 4x7x2.5mm Flanged Ball Bearing:68 ↔ RollerBearingShaft:34
- [Mate]: RollerBearingShaft:34 ↔ 4x7x2.5mm Flanged Ball Bearing:69
- [Mate]: RollerBearingShaft:34 ↔ 4x7x2.5mm Flanged Ball Bearing:69
- [Mate]: 4x7x2.5mm Flanged Ball Bearing:69 ↔ (3mm legnth) 4mm ID x 6mm OD Spacer:17
- [Mate]: 4x7x2.5mm Flanged Ball Bearing:69 ↔ (3mm legnth) 4mm ID x 6mm OD Spacer:17
- [Mate]: 4x7x2.5mm Flanged Ball Bearing:67 ↔ (3mm legnth) 4mm ID x 6mm OD Spacer:17
- [Mate]: 4x7x2.5mm Flanged Ball Bearing:67 ↔ (3mm legnth) 4mm ID x 6mm OD Spacer:17
- [Mate]: RollerBearingShaft:33 ↔ 4x7x2.5mm Flanged Ball Bearing:67
- [Mate]: RollerBearingShaft:33 ↔ 4x7x2.5mm Flanged Ball Bearing:67
- [Mate]: 4x7x2.5mm Flanged Ball Bearing:66 ↔ RollerBearingShaft:33
- [Mate]: 4x7x2.5mm Flanged Ball Bearing:66 ↔ RollerBearingShaft:33
- [Mate]: (1mm legnth) 4mm ID x 6mm OD Spacer:33 ↔ 4x7x2.5mm Flanged Ball Bearing:68
- Mate:346: HousingFaceInput:1 ↔ 4x7x2.5mm Flanged Ball Bearing:68
- [Mate]: (1mm legnth) 4mm ID x 6mm OD Spacer:35 ↔ 4x7x2.5mm Flanged Ball Bearing:72
- [Mate]: 4x7x2.5mm Flanged Ball Bearing:72 ↔ RollerBearingShaft:36
- [Mate]: 4x7x2.5mm Flanged Ball Bearing:72 ↔ RollerBearingShaft:36
- [Mate]: RollerBearingShaft:36 ↔ 4x7x2.5mm Flanged Ball Bearing:73
- [Mate]: RollerBearingShaft:36 ↔ 4x7x2.5mm Flanged Ball Bearing:73
- [Mate]: 4x7x2.5mm Flanged Ball Bearing:73 ↔ (3mm legnth) 4mm ID x 6mm OD Spacer:18
- [Mate]: 4x7x2.5mm Flanged Ball Bearing:73 ↔ (3mm legnth) 4mm ID x 6mm OD Spacer:18
- [Mate]: 4x7x2.5mm Flanged Ball Bearing:71 ↔ (3mm legnth) 4mm ID x 6mm OD Spacer:18
- [Mate]: 4x7x2.5mm Flanged Ball Bearing:71 ↔ (3mm legnth) 4mm ID x 6mm OD Spacer:18
- [Mate]: RollerBearingShaft:35 ↔ 4x7x2.5mm Flanged Ball Bearing:71
- [Mate]: RollerBearingShaft:35 ↔ 4x7x2.5mm Flanged Ball Bearing:71
- [Mate]: 4x7x2.5mm Flanged Ball Bearing:70 ↔ RollerBearingShaft:35
- [Mate]: 4x7x2.5mm Flanged Ball Bearing:70 ↔ RollerBearingShaft:35
- [Mate]: (1mm legnth) 4mm ID x 6mm OD Spacer:35 ↔ 4x7x2.5mm Flanged Ball Bearing:72
- Mate:364: HousingFaceInput:1 ↔ 4x7x2.5mm Flanged Ball Bearing:72
- [Mate]: 16mm ID x 22mm OD x 4mm Thickness Ball Bearing:3 ↔ EccentricBearingShaft:2
- Mate:372: EccentricBearingShaft:2 ↔ 16mm ID x 22mm OD x 4mm Thickness Ball Bearing:4
- Mate:373: EccentricBearingShaft:2 ↔ 16mm ID x 22mm OD x 4mm Thickness Ball Bearing:4
- Mate:374: CycloidalDisk:3 ↔ 16mm ID x 22mm OD x 4mm Thickness Ball Bearing:4
- Flush:4: CycloidalDisk:3 ↔ 16mm ID x 22mm OD x 4mm Thickness Ball Bearing:4
- Flush:5: 16mm ID x 22mm OD x 4mm Thickness Ball Bearing:3 ↔ CycloidalDisk:4
- Mate:375: 16mm ID x 22mm OD x 4mm Thickness Ball Bearing:3 ↔ CycloidalDisk:4
- Mate:377: 4x7x2.5mm Flanged Ball Bearing:6 ↔ CycloidalDisk:3
- Mate:378: 16mm ID x 22mm OD x 4mm Thickness Ball Bearing:3 ↔ EccentricBearingShaft:2
- Tangent:1: 4x7x2.5mm Flanged Ball Bearing:15 ↔ CycloidalDisk:3
- Tangent:2: 4x7x2.5mm Flanged Ball Bearing:27 ↔ CycloidalDisk:3
- Mate:379: CycloidalDisk:4 ↔ 4x7x2.5mm Flanged Ball Bearing:74
- Tangent:3: CycloidalDisk:4 ↔ 4x7x2.5mm Flanged Ball Bearing:74
- Mate:382: CycloidalDisk:3 ↔ 4x7x2.5mm Flanged Ball Bearing:75
- Tangent:4: CycloidalDisk:3 ↔ 4x7x2.5mm Flanged Ball Bearing:75
- Mate:383: 4x7x2.5mm Flanged Ball Bearing:75 ↔ (M4 x 0.7 x 16) Sockethead Buttonhead Screw:1
- Mate:384: 4x7x2.5mm Flanged Ball Bearing:75 ↔ (M4 x 0.7 x 16) Sockethead Buttonhead Screw:1
- Mate:385: 4x7x2.5mm Flanged Ball Bearing:74 ↔ (M4 x 0.7 x 16) Sockethead Buttonhead Screw:1
- Mate:386: CycloidalDisk:4 ↔ 4x7x2.5mm Flanged Ball Bearing:76
- Tangent:5: CycloidalDisk:4 ↔ 4x7x2.5mm Flanged Ball Bearing:76
- Mate:387: CycloidalDisk:3 ↔ 4x7x2.5mm Flanged Ball Bearing:77
- Tangent:6: CycloidalDisk:3 ↔ 4x7x2.5mm Flanged Ball Bearing:77
- Mate:388: 4x7x2.5mm Flanged Ball Bearing:77 ↔ (M4 x 0.7 x 16) Sockethead Buttonhead Screw:2
- Mate:389: 4x7x2.5mm Flanged Ball Bearing:77 ↔ (M4 x 0.7 x 16) Sockethead Buttonhead Screw:2
- Mate:390: 4x7x2.5mm Flanged Ball Bearing:76 ↔ (M4 x 0.7 x 16) Sockethead Buttonhead Screw:2
- Mate:391: CycloidalDisk:4 ↔ 4x7x2.5mm Flanged Ball Bearing:78
- Tangent:7: CycloidalDisk:4 ↔ 4x7x2.5mm Flanged Ball Bearing:78
- Mate:392: CycloidalDisk:4 ↔ 4x7x2.5mm Flanged Ball Bearing:79
- Mate:393: CycloidalDisk:4 ↔ 4x7x2.5mm Flanged Ball Bearing:80
- Mate:394: CycloidalDisk:4 ↔ 4x7x2.5mm Flanged Ball Bearing:81
- Tangent:8: CycloidalDisk:4 ↔ 4x7x2.5mm Flanged Ball Bearing:79
- Tangent:9: CycloidalDisk:4 ↔ 4x7x2.5mm Flanged Ball Bearing:80
- Tangent:10: CycloidalDisk:4 ↔ 4x7x2.5mm Flanged Ball Bearing:81
- Mate:395: CycloidalDisk:3 ↔ 4x7x2.5mm Flanged Ball Bearing:82
- Mate:396: CycloidalDisk:3 ↔ 4x7x2.5mm Flanged Ball Bearing:83
- Mate:397: CycloidalDisk:3 ↔ 4x7x2.5mm Flanged Ball Bearing:84
- Mate:398: CycloidalDisk:3 ↔ 4x7x2.5mm Flanged Ball Bearing:85
- Tangent:11: CycloidalDisk:3 ↔ 4x7x2.5mm Flanged Ball Bearing:82
- Tangent:12: CycloidalDisk:3 ↔ 4x7x2.5mm Flanged Ball Bearing:83
- Tangent:13: CycloidalDisk:3 ↔ 4x7x2.5mm Flanged Ball Bearing:84
- Tangent:14: CycloidalDisk:3 ↔ 4x7x2.5mm Flanged Ball Bearing:85
- Mate:399: 4x7x2.5mm Flanged Ball Bearing:85 ↔ (M4 x 0.7 x 16) Sockethead Buttonhead Screw:3
- Mate:400: 4x7x2.5mm Flanged Ball Bearing:85 ↔ (M4 x 0.7 x 16) Sockethead Buttonhead Screw:3
- Mate:401: 4x7x2.5mm Flanged Ball Bearing:84 ↔ (M4 x 0.7 x 16) Sockethead Buttonhead Screw:4
- Mate:402: 4x7x2.5mm Flanged Ball Bearing:84 ↔ (M4 x 0.7 x 16) Sockethead Buttonhead Screw:4
- Mate:403: 4x7x2.5mm Flanged Ball Bearing:83 ↔ (M4 x 0.7 x 16) Sockethead Buttonhead Screw:5
- Mate:404: 4x7x2.5mm Flanged Ball Bearing:83 ↔ (M4 x 0.7 x 16) Sockethead Buttonhead Screw:5
- Mate:405: 4x7x2.5mm Flanged Ball Bearing:82 ↔ (M4 x 0.7 x 16) Sockethead Buttonhead Screw:6
- Mate:406: 4x7x2.5mm Flanged Ball Bearing:82 ↔ (M4 x 0.7 x 16) Sockethead Buttonhead Screw:6
- Mate:407: 4x7x2.5mm Flanged Ball Bearing:81 ↔ (M4 x 0.7 x 16) Sockethead Buttonhead Screw:6
- Mate:408: 4x7x2.5mm Flanged Ball Bearing:78 ↔ (M4 x 0.7 x 16) Sockethead Buttonhead Screw:3
- Mate:409: 4x7x2.5mm Flanged Ball Bearing:79 ↔ (M4 x 0.7 x 16) Sockethead Buttonhead Screw:4
- Mate:410: 4x7x2.5mm Flanged Ball Bearing:80 ↔ (M4 x 0.7 x 16) Sockethead Buttonhead Screw:5
- Tangent:15: 4x7x2.5mm Flanged Ball Bearing:72 ↔ CycloidalDisk:4
- Mate:411: 4x7x2.5mm Flanged Ball Bearing:22 ↔ HousingInputFaceSpacer:1
- Mate:412: 4x7x2.5mm Flanged Ball Bearing:22 ↔ HousingInputFaceSpacer:1
- Mate:413: 4x7x2.5mm Flanged Ball Bearing:26 ↔ HousingInputFaceSpacer:2
- Mate:414: 4x7x2.5mm Flanged Ball Bearing:26 ↔ HousingInputFaceSpacer:2
- Mate:415: 4x7x2.5mm Flanged Ball Bearing:30 ↔ HousingInputFaceSpacer:3
- Mate:416: 4x7x2.5mm Flanged Ball Bearing:30 ↔ HousingInputFaceSpacer:3
- Mate:417: 4x7x2.5mm Flanged Ball Bearing:34 ↔ HousingInputFaceSpacer:4
- Mate:418: 4x7x2.5mm Flanged Ball Bearing:34 ↔ HousingInputFaceSpacer:4
- Mate:419: 4x7x2.5mm Flanged Ball Bearing:38 ↔ HousingInputFaceSpacer:5
- Mate:420: 4x7x2.5mm Flanged Ball Bearing:38 ↔ HousingInputFaceSpacer:5
- Mate:421: 4x7x2.5mm Flanged Ball Bearing:42 ↔ HousingInputFaceSpacer:6
- Mate:422: 4x7x2.5mm Flanged Ball Bearing:42 ↔ HousingInputFaceSpacer:6
- Mate:423: 4x7x2.5mm Flanged Ball Bearing:46 ↔ HousingInputFaceSpacer:7
- Mate:424: 4x7x2.5mm Flanged Ball Bearing:46 ↔ HousingInputFaceSpacer:7
- Mate:425: 4x7x2.5mm Flanged Ball Bearing:50 ↔ HousingInputFaceSpacer:8
- Mate:426: 4x7x2.5mm Flanged Ball Bearing:50 ↔ HousingInputFaceSpacer:8
- Mate:427: 4x7x2.5mm Flanged Ball Bearing:54 ↔ HousingInputFaceSpacer:9
- Mate:428: 4x7x2.5mm Flanged Ball Bearing:54 ↔ HousingInputFaceSpacer:9
- Mate:429: 4x7x2.5mm Flanged Ball Bearing:58 ↔ HousingInputFaceSpacer:10
- Mate:430: 4x7x2.5mm Flanged Ball Bearing:58 ↔ HousingInputFaceSpacer:10
- Mate:431: 4x7x2.5mm Flanged Ball Bearing:62 ↔ HousingInputFaceSpacer:11
- Mate:432: 4x7x2.5mm Flanged Ball Bearing:62 ↔ HousingInputFaceSpacer:11
- Mate:433: 4x7x2.5mm Flanged Ball Bearing:66 ↔ HousingInputFaceSpacer:12
- Mate:434: 4x7x2.5mm Flanged Ball Bearing:66 ↔ HousingInputFaceSpacer:12
- Mate:435: 4x7x2.5mm Flanged Ball Bearing:70 ↔ HousingInputFaceSpacer:13
- Mate:436: 4x7x2.5mm Flanged Ball Bearing:70 ↔ HousingInputFaceSpacer:13
## Named parameters: d439_d394 = 0 mm, d440_d349 = 0 mm, d441_d350 = 0 mm, d442_d351 = 0 mm, d443_d352 = 0 mm, d444_d353 = 0 mm, d447_d340 = 0 mm, d448_d342 = 0 mm, d449_d343 = 0 mm, d450_d344 = 0 mm, d451_d345 = 0 mm, d452_d346 = 0 mm, d453_d347 = 0 mm, d454_d348 = 0 mm, d457_d394 = 0 mm, d458_d349 = 0 mm, d459_d350 = 0 mm, d460_d351 = 0 mm, d461_d352 = 0 mm, d462_d353 = 0 mm, d465_d340 = 0 mm, d466_d342 = 0 mm, d467_d343 = 0 mm, d468_d344 = 0 mm, d469_d345 = 0 mm, d470_d346 = 0 mm, d471_d347 = 0 mm, d472_d348 = 0 mm, d475_d394 = 0 mm, d476_d349 = 0 mm, d477_d350 = 0 mm, d478_d351 = 0 mm, d479_d352 = 0 mm, d480_d353 = 0 mm, d483_d340 = 0 mm, d484_d342 = 0 mm, d485_d343 = 0 mm, d486_d344 = 0 mm, d487_d345 = 0 mm, d488_d346 = 0 mm, d489_d347 = 0 mm, d490_d348 = 0 mm, d493_d394 = 0 mm, d494_d349 = 0 mm, d495_d350 = 0 mm, d496_d351 = 0 mm, d497_d352 = 0 mm, d498_d353 = 0 mm, d501_d340 = 0 mm, d502_d342 = 0 mm, d503_d343 = 0 mm, d504_d344 = 0 mm, d505_d345 = 0 mm, d506_d346 = 0 mm, d507_d347 = 0 mm, d508_d348 = 0 mm, d511_d394 = 0 mm, d512_d349 = 0 mm, d513_d350 = 0 mm, d514_d351 = 0 mm, d515_d352 = 0 mm, d516_d353 = 0 mm, d519_d340 = 0 mm, d520_d342 = 0 mm, d521_d343 = 0 mm, d522_d344 = 0 mm, d523_d345 = 0 mm, d524_d346 = 0 mm, d525_d347 = 0 mm, d526_d348 = 0 mm, d529_d394 = 0 mm, d530_d349 = 0 mm, d531_d350 = 0 mm, d532_d351 = 0 mm, d533_d352 = 0 mm, d534_d353 = 0 mm, d537_d340 = 0 mm, d538_d342 = 0 mm, d539_d343 = 0 mm, d540_d344 = 0 mm, d541_d345 = 0 mm, d542_d346 = 0 mm, d543_d347 = 0 mm, d544_d348 = 0 mm, d547_d394 = 0 mm, d548_d349 = 0 mm, d549_d350 = 0 mm, d550_d351 = 0 mm, d551_d352 = 0 mm, d552_d353 = 0 mm, d555_d340 = 0 mm, d556_d342 = 0 mm, d557_d343 = 0 mm, d558_d344 = 0 mm, d559_d345 = 0 mm, d560_d346 = 0 mm, d561_d347 = 0 mm, d562_d348 = 0 mm, d565_d394 = 0 mm, d566_d349 = 0 mm, d567_d350 = 0 mm, d568_d351 = 0 mm, d569_d352 = 0 mm, d570_d353 = 0 mm, d573_d340 = 0 mm, d574_d342 = 0 mm, d575_d343 = 0 mm, d576_d344 = 0 mm, d577_d345 = 0 mm, d578_d346 = 0 mm, d579_d347 = 0 mm, d580_d348 = 0 mm, d583_d394 = 0 mm, d584_d349 = 0 mm, d585_d350 = 0 mm, d586_d351 = 0 mm, d587_d352 = 0 mm, d588_d353 = 0 mm, d591_d340 = 0 mm, d592_d342 = 0 mm, d593_d343 = 0 mm, d594_d344 = 0 mm, d595_d345 = 0 mm, d596_d346 = 0 mm, d597_d347 = 0 mm, d598_d348 = 0 mm, d601_d394 = 0 mm, d602_d349 = 0 mm, d603_d350 = 0 mm, d604_d351 = 0 mm, d605_d352 = 0 mm, d606_d353 = 0 mm, d609_d340 = 0 mm, d610_d342 = 0 mm, d611_d343 = 0 mm, d612_d344 = 0 mm, d613_d345 = 0 mm, d614_d346 = 0 mm, d615_d347 = 0 mm, d616_d348 = 0 mm, d619_d394 = 0 mm, d620_d349 = 0 mm, d621_d350 = 0 mm, d622_d351 = 0 mm, d623_d352 = 0 mm, d624_d353 = 0 mm, d627_d340 = 0 mm, d628_d342 = 0 mm, d629_d343 = 0 mm, d630_d344 = 0 mm, d631_d345 = 0 mm, d632_d346 = 0 mm, d633_d347 = 0 mm, d634_d348 = 0 mm, d637_d394 = 0 mm, d638_d349 = 0 mm, d639_d350 = 0 mm, d640_d351 = 0 mm, d641_d352 = 0 mm, d642_d353 = 0 mm, d645_d340 = 0 mm, d646_d342 = 0 mm, d647_d343 = 0 mm, d648_d344 = 0 mm, d649_d345 = 0 mm, d650_d346 = 0 mm, d651_d347 = 0 mm, d652_d348 = 0 mm, d655_d394 = 0 mm, d656_d349 = 0 mm, d657_d350 = 0 mm, d658_d351 = 0 mm, d659_d352 = 0 mm, d660_d353 = 0 mm, d663_d340 = 0 mm, d664_d342 = 0 mm, d665_d343 = 0 mm, d666_d344 = 0 mm, d667_d345 = 0 mm, d668_d346 = 0 mm, d669_d347 = 0 mm, d670_d348 = 0 mm, d673_d394 = 0 mm, d674_d349 = 0 mm, d675_d350 = 0 mm, d676_d351 = 0 mm, d677_d352 = 0 mm, d678_d353 = 0 mm, d681_d340 = 0 mm, d682_d342 = 0 mm, d683_d343 = 0 mm, d684_d344 = 0 mm, d685_d345 = 0 mm, d686_d346 = 0 mm, d687_d347 = 0 mm, d688_d348 = 0 mm, d691_d394 = 0 mm, d692_d349 = 0 mm, d693_d350 = 0 mm, d694_d351 = 0 mm, d695_d352 = 0 mm, d696_d353 = 0 mm, d699_d340 = 0 mm, d700_d342 = 0 mm, d701_d343 = 0 mm, d702_d344 = 0 mm, d703_d345 = 0 mm, d704_d346 = 0 mm, d705_d347 = 0 mm, d706_d348 = 0 mm, d709_d394 = 0 mm, d710_d349 = 0 mm, d711_d350 = 0 mm, d712_d351 = 0 mm, d713_d352 = 0 mm, d714_d353 = 0 mm, d717_d340 = 0 mm, d718_d342 = 0 mm, d719_d343 = 0 mm, d720_d344 = 0 mm, d721_d345 = 0 mm, d722_d346 = 0 mm, d723_d347 = 0 mm, d724_d348 = 0 mm, d727_d394 = 0 mm, d728_d349 = 0 mm, d729_d350 = 0 mm, d730_d351 = 0 mm, d731_d352 = 0 mm, d732_d353 = 0 mm, d735_d340 = 0 mm, d736_d342 = 0 mm, d737_d343 = 0 mm, d738_d344 = 0 mm, d739_d345 = 0 mm, d740_d346 = 0 mm, d741_d347 = 0 mm, d742_d348 = 0 mm, d767_d763 = 0 mm
